# Autodesk Inventor assembly: CAR_015_NewCarouselTensionerAssembly
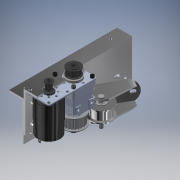
[picture p0: Inventor's stored thumbnail of the model, 180x180]
Saved by Autodesk Inventor 2018.3 (Build 223284000, 284)
## iProperties
Created: 2020-02-01
Part Number: CAR_015_NewCarouselTensionerAssembly
Document SubType Name: Assembly
Designer: user
Mass: 211.586 g
Surface Area: 527.901 cm^2
Volume: 81.806 cm^3
Density: 2.58644 g/cm^3
Author: user
## Documents named in this file (6)
- C:\Users\22barlalex\Documents\GrabCAD\Infinite Recharge 2020\Build season\CAR_015_NewCarouselTensionerAssembly.iam
- C:\Users\22barlalex\Documents\GrabCAD\Infinite Recharge 2020\Build season\CAR_019_TensionerLBracket_MIR.ipt
- C:\Users\22barlalex\Documents\GrabCAD\Infinite Recharge 2020\Build season\CAR_012_CarouselDriveAssembly.iam
- C:\Users\22barlalex\Documents\GrabCAD\Infinite Recharge 2020\Build season\CAR_033_CarouselBelt.ipt
- C:\Users\22barlalex\Documents\GrabCAD\Infinite Recharge 2020\Build season\CAR_044_180VersaLBracketMount.ipt
- C:\Users\22barlalex\Documents\GrabCAD\Infinite Recharge 2020\Build season\CAR_046_NewCarouselTensioner.iam
## Components (5 placed, 5 different names)
1. CAR_019_TensionerLBracket_MIR:1 — Mate:5, Mate:6, Angle:1, Mate:9, Mate:10, Mate:16
2. CAR_012_CarouselDriveAssembly:1 [sub-assembly] — Mate:5, Mate:6, Mate:7, Mate:9, Mate:11, Flush:5, Mate:12, Flush:14
3. CAR_033_CarouselBelt:1 — Mate:7, Angle:1, Mate:8, Flush:4
4. CAR_044_180VersaLBracketMount:1 — Mate:10, Mate:11, Flush:5, Mate:15
5. CAR_046_NewCarouselTensioner:1 [sub-assembly] — Flush:14, Mate:15, Mate:16
## Relationships (14: Mate 10, Flush 3, Angle 1)
- Mate:5: CAR_019_TensionerLBracket_MIR:1 ↔ CAR_012_CarouselDriveAssembly:1
- Mate:6: CAR_019_TensionerLBracket_MIR:1 ↔ CAR_012_CarouselDriveAssembly:1
- Mate:7: CAR_012_CarouselDriveAssembly:1 ↔ CAR_033_CarouselBelt:1
- Angle:1 (0 deg): CAR_019_TensionerLBracket_MIR:1 ↔ CAR_033_CarouselBelt:1
- Mate:8: CAR_033_CarouselBelt:1
- Flush:4: CAR_033_CarouselBelt:1
- Mate:9 (3.175 mm): CAR_019_TensionerLBracket_MIR:1 ↔ CAR_012_CarouselDriveAssembly:1
- Mate:10: CAR_019_TensionerLBracket_MIR:1 ↔ CAR_044_180VersaLBracketMount:1
- Mate:11: CAR_012_CarouselDriveAssembly:1 ↔ CAR_044_180VersaLBracketMount:1
- Flush:5: CAR_012_CarouselDriveAssembly:1 ↔ CAR_044_180VersaLBracketMount:1
- Mate:12: CAR_012_CarouselDriveAssembly:1
- Flush:14: CAR_012_CarouselDriveAssembly:1 ↔ CAR_046_NewCarouselTensioner:1
- Mate:15 (6.35 mm): CAR_044_180VersaLBracketMount:1 ↔ CAR_046_NewCarouselTensioner:1
- Mate:16: CAR_019_TensionerLBracket_MIR:1 ↔ CAR_046_NewCarouselTensioner:1
